# Autodesk Inventor assembly: 000.001 - Ходовая часть
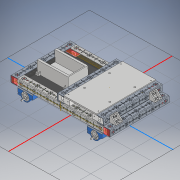
[picture p0: Inventor's stored thumbnail of the model, 180x180]
Saved by Autodesk Inventor 2022 (Build 260153000, 153)
## iProperties
Created: 2022-01-16
Part Number: 000.001 - Ходовая часть
Document SubType Name: Assembly
Designer: Петров Иван
Author: Петров Иван
## Documents named in this file (17)
- D:\IVAN\Ivan_desktop\Kvantorium\Projects\YouBotRobot\design\000.001 - Ходовая часть.iam
- D:\IVAN\Ivan_desktop\Kvantorium\Projects\YouBotRobot\design\standart_components\Tetrix\ftc-tetrix-kit-of-parts-1.snapshot.34\MAX Channels\416mm Channel.ipt
- D:\IVAN\Ivan_desktop\Kvantorium\Projects\YouBotRobot\design\standart_components\Tetrix\Tetrix_Kit_FTC\tetrix_288mm_channel.ipt
- D:\IVAN\Ivan_desktop\Kvantorium\Projects\YouBotRobot\design\000.001.001 - Уголок.ipt
- D:\IVAN\Ivan_desktop\Kvantorium\Projects\YouBotRobot\design\000.002 - Крепеж мотора СБ.iam
- D:\IVAN\Ivan_desktop\Kvantorium\Projects\YouBotRobot\design\000.001.002 - Днище.ipt
- D:\IVAN\Ivan_desktop\Kvantorium\Projects\YouBotRobot\design\standart_components\JetsonNano\Jetson nano_fixed.iam
- D:\IVAN\Ivan_desktop\Kvantorium\Projects\YouBotRobot\design\standart_components\Raspberry Pi 4B\Raspberry-Pi-4-Model-B-03.ipt
- D:\IVAN\Ivan_desktop\Kvantorium\Projects\YouBotRobot\design\standart_components\L298N\L298N_V2.ipt
- D:\IVAN\Ivan_desktop\Kvantorium\Projects\YouBotRobot\design\standart_components\TPlinkTL-SF1008D.ipt
- D:\IVAN\Ivan_desktop\Kvantorium\Projects\YouBotRobot\design\000.001.003 - Уголок.ipt
- D:\IVAN\Ivan_desktop\Kvantorium\Projects\YouBotRobot\design\000.001.004 - Держатель для проводов.ipt
- D:\IVAN\Ivan_desktop\Kvantorium\Projects\YouBotRobot\electronic\jetson_power_board\untitled.brd.iam
- D:\IVAN\Ivan_desktop\Kvantorium\Projects\YouBotRobot\design\000.003 - Блок АКБ СБ.iam
- D:\IVAN\Ivan_desktop\Kvantorium\Projects\YouBotRobot\design\000.001.004 - Уголок.ipt
- D:\IVAN\Ivan_desktop\Kvantorium\Projects\YouBotRobot\design\000.001.006 - Площадка под манипулятор.ipt
- D:\IVAN\Ivan_desktop\Kvantorium\Projects\BaumanBot\Днище.ipt
## Components (37 placed, 16 different names)
1. 416mm Channel:1 — Совмещение:27, Совмещение:52, Заподлицо:1, Заподлицо:2, Совмещение:59, Совмещение:65, Совмещение:66, Совмещение:67, Совмещение:68, Совмещение:70, Совмещение:71, Совмещение:80, Совмещение:81, Совмещение:82, Совмещение:83, Совмещение:84, Совмещение:85, Совмещение:97, Совмещение:100, Совмещение:105
2. 416mm Channel:2 — Заподлицо:3, Заподлицо:4, Совмещение:53, Заподлицо:5, Заподлицо:6, Совмещение:54, Совмещение:55, Совмещение:56, Совмещение:57, Совмещение:62, Совмещение:69, Совмещение:74, Совмещение:76, Совмещение:77, Совмещение:78, Совмещение:79, Совмещение:88, Совмещение:91, Совмещение:94, Совмещение:103, Совмещение:104
3. tetrix_288mm_channel:1 — Совмещение:51, Заподлицо:5, Заподлицо:6, Совмещение:54, Совмещение:63, Совмещение:64, Совмещение:90
4. tetrix_288mm_channel:2 — Совмещение:52, Заподлицо:1, Заподлицо:2, Заподлицо:3, Заподлицо:4, Совмещение:53, Совмещение:58, Совмещение:60, Совмещение:61, Совмещение:75, Совмещение:138, Совмещение:139, Совмещение:140, Совмещение:141
5. 000.001.001 - Уголок:1 — Совмещение:55, Совмещение:56, Совмещение:57, Совмещение:58
6. 000.001.001 - Уголок:2 — Совмещение:59, Совмещение:60, Совмещение:61
7. 000.001.001 - Уголок:3 — Совмещение:62, Совмещение:63, Совмещение:64
8. 000.001.001 - Уголок:4 — Совмещение:65, Совмещение:66, Совмещение:67
9. tetrix_288mm_channel:3 — Совмещение:68, Совмещение:69, Совмещение:70, Совмещение:93, Совмещение:96, Совмещение:109, Совмещение:110, Совмещение:111, Совмещение:118, Совмещение:119, Совмещение:120, Угол:1, Совмещение:142, Совмещение:143
10. tetrix_288mm_channel:4 — Совмещение:71, Совмещение:101, Совмещение:102, Совмещение:104, Совмещение:105, Совмещение:112, Совмещение:113, Совмещение:114, Совмещение:115, Совмещение:116, Совмещение:117, Совмещение:121, Совмещение:122, Заподлицо:9
11. 000.002 - Крепеж мотора СБ:1 [sub-assembly] — Совмещение:74, Совмещение:75, Совмещение:76, Касательность:1
12. 000.002 - Крепеж мотора СБ:2 [sub-assembly] — Совмещение:77, Совмещение:78, Совмещение:79
13. 000.002 - Крепеж мотора СБ:3 [sub-assembly] — Совмещение:80, Совмещение:81, Совмещение:82
14. 000.002 - Крепеж мотора СБ:4 [sub-assembly] — Совмещение:83, Совмещение:84, Совмещение:85
15. 000.001.002 - Днище:1 — Совмещение:88, Совмещение:90, Совмещение:91, Совмещение:92, Совмещение:95, Совмещение:98, Совмещение:99, Совмещение:124, Совмещение:125, Совмещение:126, Совмещение:127, Совмещение:128, Совмещение:129, Совмещение:130, Совмещение:131, Совмещение:132, Совмещение:133, Совмещение:134, Совмещение:136
16. Jetson nano_fixed:1 [sub-assembly] — Совмещение:92, Совмещение:93, Совмещение:94
17. Raspberry-Pi-4-Model-B-03:1 — Совмещение:95, Совмещение:96, Совмещение:97
18. L298N_V2:1 — Совмещение:98, Совмещение:100, Совмещение:101, Угол:2
19. L298N_V2:2 — Совмещение:99, Совмещение:102, Совмещение:103, Угол:4
20. TPlinkTL-SF1008D:1 — Совмещение:121, Совмещение:122, Совмещение:123
21. 000.001.003 - Уголок:1 — Совмещение:109, Совмещение:110, Совмещение:111
22. 000.001.003 - Уголок:2 — Совмещение:112, Совмещение:113, Совмещение:114, Совмещение:123
23. 000.001.003 - Уголок:3 — Совмещение:115, Совмещение:116, Совмещение:117
24. 000.001.003 - Уголок:4 — Совмещение:118, Совмещение:119, Совмещение:120, Совмещение:144
25. 000.001.004 - Держатель для проводов:4 — Совмещение:126, Совмещение:127, Угол:2, Угол:3
26. 000.001.004 - Держатель для проводов:5 — Совмещение:128, Совмещение:129, Угол:3
27. 000.001.004 - Держатель для проводов:6 — Совмещение:130, Совмещение:131, Угол:4, Угол:5
28. 000.001.004 - Держатель для проводов:7 — Совмещение:132, Совмещение:133, Угол:5, Заподлицо:8, Совмещение:137
29. untitled.brd:1 [sub-assembly] — Совмещение:134, Совмещение:135, Заподлицо:7
30. 000.003 - Блок АКБ СБ:1 [sub-assembly] — Совмещение:136, Заподлицо:8, Совмещение:137
31. 000.001.004 - Уголок:1 — Совмещение:138, Совмещение:139
32. 000.001.004 - Уголок:2 — Совмещение:140, Совмещение:141, Совмещение:142
33. 000.001.006 - Площадка под манипулятор:1 — Совмещение:143, Заподлицо:9, Совмещение:144, Совмещение:145, Совмещение:146, Угол:6
34. Днище:1 — Совмещение:145, Совмещение:146, Угол:6
35. 000.001.004 - Держатель для проводов:1 — Совмещение:124, Совмещение:125, Угол:1
36. 000.001.004 - Держатель для проводов:2
37. 000.001.004 - Держатель для проводов:3 — Совмещение:135, Заподлицо:7
## Component patterns: (3 elements, first: 000.001.004 - Держатель для проводов:1)
## Relationships (105: Mate 89, Flush 9, Angle 6, Tangent 1)
- Совмещение:27 [Mate]: 416mm Channel:1
- Совмещение:51 [Mate]: tetrix_288mm_channel:1
- Совмещение:52 [Mate]: 416mm Channel:1 ↔ tetrix_288mm_channel:2
- Заподлицо:1 [Flush]: 416mm Channel:1 ↔ tetrix_288mm_channel:2
- Заподлицо:2 [Flush]: 416mm Channel:1 ↔ tetrix_288mm_channel:2
- Заподлицо:3 [Flush]: 416mm Channel:2 ↔ tetrix_288mm_channel:2
- Заподлицо:4 [Flush]: 416mm Channel:2 ↔ tetrix_288mm_channel:2
- Совмещение:53 [Mate]: 416mm Channel:2 ↔ tetrix_288mm_channel:2
- Заподлицо:5 [Flush]: 416mm Channel:2 ↔ tetrix_288mm_channel:1
- Заподлицо:6 [Flush]: 416mm Channel:2 ↔ tetrix_288mm_channel:1
- Совмещение:54 [Mate]: 416mm Channel:2 ↔ tetrix_288mm_channel:1
- Совмещение:55 [Mate]: 416mm Channel:2 ↔ 000.001.001 - Уголок:1
- Совмещение:56 [Mate]: 416mm Channel:2 ↔ 000.001.001 - Уголок:1
- Совмещение:57 [Mate]: 416mm Channel:2 ↔ 000.001.001 - Уголок:1
- Совмещение:58 [Mate]: tetrix_288mm_channel:2 ↔ 000.001.001 - Уголок:1
- Совмещение:59 [Mate]: 416mm Channel:1 ↔ 000.001.001 - Уголок:2
- Совмещение:60 [Mate]: tetrix_288mm_channel:2 ↔ 000.001.001 - Уголок:2
- Совмещение:61 [Mate]: tetrix_288mm_channel:2 ↔ 000.001.001 - Уголок:2
- Совмещение:62 [Mate]: 416mm Channel:2 ↔ 000.001.001 - Уголок:3
- Совмещение:63 [Mate]: tetrix_288mm_channel:1 ↔ 000.001.001 - Уголок:3
- Совмещение:64 [Mate]: tetrix_288mm_channel:1 ↔ 000.001.001 - Уголок:3
- Совмещение:65 [Mate]: 416mm Channel:1 ↔ 000.001.001 - Уголок:4
- Совмещение:66 [Mate]: 416mm Channel:1 ↔ 000.001.001 - Уголок:4
- Совмещение:67 [Mate]: 416mm Channel:1 ↔ 000.001.001 - Уголок:4
- Совмещение:68 [Mate]: 416mm Channel:1 ↔ tetrix_288mm_channel:3
- Совмещение:69 [Mate]: 416mm Channel:2 ↔ tetrix_288mm_channel:3
- Совмещение:70 [Mate]: 416mm Channel:1 ↔ tetrix_288mm_channel:3
- Совмещение:71 [Mate]: 416mm Channel:1 ↔ tetrix_288mm_channel:4
- Совмещение:74 [Mate]: 416mm Channel:2 ↔ 000.002 - Крепеж мотора СБ:1
- Совмещение:75 [Mate] (4 mm): tetrix_288mm_channel:2 ↔ 000.002 - Крепеж мотора СБ:1
- Совмещение:76 [Mate]: 416mm Channel:2 ↔ 000.002 - Крепеж мотора СБ:1
- Совмещение:77 [Mate]: 416mm Channel:2 ↔ 000.002 - Крепеж мотора СБ:2
- Совмещение:78 [Mate]: 416mm Channel:2 ↔ 000.002 - Крепеж мотора СБ:2
- Совмещение:79 [Mate]: 416mm Channel:2 ↔ 000.002 - Крепеж мотора СБ:2
- Совмещение:80 [Mate]: 416mm Channel:1 ↔ 000.002 - Крепеж мотора СБ:3
- Совмещение:81 [Mate]: 416mm Channel:1 ↔ 000.002 - Крепеж мотора СБ:3
- Совмещение:82 [Mate]: 416mm Channel:1 ↔ 000.002 - Крепеж мотора СБ:3
- Совмещение:83 [Mate]: 416mm Channel:1 ↔ 000.002 - Крепеж мотора СБ:4
- Совмещение:84 [Mate]: 416mm Channel:1 ↔ 000.002 - Крепеж мотора СБ:4
- Совмещение:85 [Mate]: 416mm Channel:1 ↔ 000.002 - Крепеж мотора СБ:4
- Совмещение:88 [Mate]: 416mm Channel:2 ↔ 000.001.002 - Днище:1
- Совмещение:90 [Mate]: tetrix_288mm_channel:1 ↔ 000.001.002 - Днище:1
- Совмещение:91 [Mate]: 416mm Channel:2 ↔ 000.001.002 - Днище:1
- Совмещение:92 [Mate] (5 mm): 000.001.002 - Днище:1 ↔ Jetson nano_fixed:1
- Совмещение:93 [Mate]: tetrix_288mm_channel:3 ↔ Jetson nano_fixed:1
- Совмещение:94 [Mate] (5 mm): 416mm Channel:2 ↔ Jetson nano_fixed:1
- Совмещение:95 [Mate] (5 mm): 000.001.002 - Днище:1 ↔ Raspberry-Pi-4-Model-B-03:1
- Совмещение:96 [Mate]: tetrix_288mm_channel:3 ↔ Raspberry-Pi-4-Model-B-03:1
- Совмещение:97 [Mate] (10 mm): 416mm Channel:1 ↔ Raspberry-Pi-4-Model-B-03:1
- Совмещение:98 [Mate] (5 mm): 000.001.002 - Днище:1 ↔ L298N_V2:1
- Совмещение:99 [Mate] (5 mm): 000.001.002 - Днище:1 ↔ L298N_V2:2
- Совмещение:100 [Mate] (4 mm): 416mm Channel:1 ↔ L298N_V2:1
- Совмещение:101 [Mate] (15 mm): tetrix_288mm_channel:4 ↔ L298N_V2:1
- Совмещение:102 [Mate] (15 mm): tetrix_288mm_channel:4 ↔ L298N_V2:2
- Совмещение:103 [Mate] (4 mm): 416mm Channel:2 ↔ L298N_V2:2
- Совмещение:104 [Mate]: 416mm Channel:2 ↔ tetrix_288mm_channel:4
- Совмещение:105 [Mate]: 416mm Channel:1 ↔ tetrix_288mm_channel:4
- Совмещение:109 [Mate]: tetrix_288mm_channel:3 ↔ 000.001.003 - Уголок:1
- Совмещение:110 [Mate]: tetrix_288mm_channel:3 ↔ 000.001.003 - Уголок:1
- Совмещение:111 [Mate]: tetrix_288mm_channel:3 ↔ 000.001.003 - Уголок:1
- Совмещение:112 [Mate]: tetrix_288mm_channel:4 ↔ 000.001.003 - Уголок:2
- Совмещение:113 [Mate]: tetrix_288mm_channel:4 ↔ 000.001.003 - Уголок:2
- Совмещение:114 [Mate]: tetrix_288mm_channel:4 ↔ 000.001.003 - Уголок:2
- Совмещение:115 [Mate]: tetrix_288mm_channel:4 ↔ 000.001.003 - Уголок:3
- Совмещение:116 [Mate]: tetrix_288mm_channel:4 ↔ 000.001.003 - Уголок:3
- Совмещение:117 [Mate]: tetrix_288mm_channel:4 ↔ 000.001.003 - Уголок:3
- Совмещение:118 [Mate]: tetrix_288mm_channel:3 ↔ 000.001.003 - Уголок:4
- Совмещение:119 [Mate]: tetrix_288mm_channel:3 ↔ 000.001.003 - Уголок:4
- Совмещение:120 [Mate]: tetrix_288mm_channel:3 ↔ 000.001.003 - Уголок:4
- Совмещение:121 [Mate]: tetrix_288mm_channel:4 ↔ TPlinkTL-SF1008D:1
- Совмещение:122 [Mate]: tetrix_288mm_channel:4 ↔ TPlinkTL-SF1008D:1
- Совмещение:123 [Mate] (40 mm): TPlinkTL-SF1008D:1 ↔ 000.001.003 - Уголок:2
- Совмещение:124 [Mate]: 000.001.002 - Днище:1 ↔ 000.001.004 - Держатель для проводов:1
- Совмещение:125 [Mate]: 000.001.002 - Днище:1 ↔ 000.001.004 - Держатель для проводов:1
- Угол:1 [Angle] (0 deg): tetrix_288mm_channel:3 ↔ 000.001.004 - Держатель для проводов:1
- Совмещение:126 [Mate]: 000.001.002 - Днище:1 ↔ 000.001.004 - Держатель для проводов:4
- Совмещение:127 [Mate]: 000.001.002 - Днище:1 ↔ 000.001.004 - Держатель для проводов:4
- Угол:2 [Angle] (0 deg): L298N_V2:1 ↔ 000.001.004 - Держатель для проводов:4
- Совмещение:128 [Mate]: 000.001.002 - Днище:1 ↔ 000.001.004 - Держатель для проводов:5
- Совмещение:129 [Mate]: 000.001.002 - Днище:1 ↔ 000.001.004 - Держатель для проводов:5
- Угол:3 [Angle] (0 deg): 000.001.004 - Держатель для проводов:4 ↔ 000.001.004 - Держатель для проводов:5
- Совмещение:130 [Mate]: 000.001.002 - Днище:1 ↔ 000.001.004 - Держатель для проводов:6
- Совмещение:131 [Mate]: 000.001.002 - Днище:1 ↔ 000.001.004 - Держатель для проводов:6
- Угол:4 [Angle] (0 deg): L298N_V2:2 ↔ 000.001.004 - Держатель для проводов:6
- Совмещение:132 [Mate]: 000.001.002 - Днище:1 ↔ 000.001.004 - Держатель для проводов:7
- Совмещение:133 [Mate]: 000.001.002 - Днище:1 ↔ 000.001.004 - Держатель для проводов:7
- Угол:5 [Angle] (0 deg): 000.001.004 - Держатель для проводов:6 ↔ 000.001.004 - Держатель для проводов:7
- Совмещение:134 [Mate] (5 mm): 000.001.002 - Днище:1 ↔ untitled.brd:1
- Совмещение:135 [Mate] (10 mm): untitled.brd:1 ↔ 000.001.004 - Держатель для проводов:3
- Заподлицо:7 [Flush]: untitled.brd:1 ↔ 000.001.004 - Держатель для проводов:3
- Совмещение:136 [Mate]: 000.001.002 - Днище:1 ↔ 000.003 - Блок АКБ СБ:1
- Заподлицо:8 [Flush]: 000.001.004 - Держатель для проводов:7 ↔ 000.003 - Блок АКБ СБ:1
- Совмещение:137 [Mate]: 000.001.004 - Держатель для проводов:7 ↔ 000.003 - Блок АКБ СБ:1
- Совмещение:138 [Mate]: tetrix_288mm_channel:2 ↔ 000.001.004 - Уголок:1
- Совмещение:139 [Mate]: tetrix_288mm_channel:2 ↔ 000.001.004 - Уголок:1
- Совмещение:140 [Mate]: tetrix_288mm_channel:2 ↔ 000.001.004 - Уголок:2
- Совмещение:141 [Mate]: tetrix_288mm_channel:2 ↔ 000.001.004 - Уголок:2
- Совмещение:142 [Mate]: tetrix_288mm_channel:3 ↔ 000.001.004 - Уголок:2
- Совмещение:143 [Mate]: tetrix_288mm_channel:3 ↔ 000.001.006 - Площадка под манипулятор:1
- Заподлицо:9 [Flush]: tetrix_288mm_channel:4 ↔ 000.001.006 - Площадка под манипулятор:1
- Совмещение:144 [Mate]: 000.001.003 - Уголок:4 ↔ 000.001.006 - Площадка под манипулятор:1
- Совмещение:145 [Mate]: 000.001.006 - Площадка под манипулятор:1 ↔ Днище:1
- Совмещение:146 [Mate]: 000.001.006 - Площадка под манипулятор:1 ↔ Днище:1
- Угол:6 [Angle] (0 deg): 000.001.006 - Площадка под манипулятор:1 ↔ Днище:1
- Касательность:1 [Tangent]: 000.002 - Крепеж мотора СБ:1
